# Autodesk Inventor assembly: circuit_boule
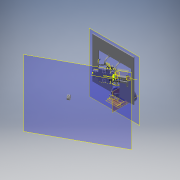
[picture p0: Inventor's stored thumbnail of the model, 180x180]
Saved by Autodesk Inventor 2017 (Build 210142000, 142)
## iProperties
Part Number: circuit_boule
Material: Générique
Document SubType Name: Assembly
Designer: Thomas
Author: Thomas
## Documents named in this file (7)
- C:\Users\Thomas\Documents\Modele 3D\Lanceur boule\circuit_boule.iam
- C:\Users\Thomas\Documents\Modele 3D\Lanceur boule\conduit.ipt
- C:\Users\Thomas\Documents\Modele 3D\Lanceur boule\conduit_bis.ipt
- C:\Users\Thomas\Documents\Modele 3D\Lanceur boule\anneau.ipt
- C:\Users\Thomas\Documents\Modele 3D\Lanceur boule\anneau2.ipt
- C:\Users\Thomas\Documents\Modele 3D\Lanceur boule\Plaque vois.ipt
- C:\Users\Thomas\Documents\Modele 3D\Lanceur boule\Ensemble_Lanceur.iam
## Components (9 placed, 6 different names)
1. conduit:1 — Placage:2, Placage:3
2. conduit_bis:1 — Placage:2, Placage:3
3. anneau:1 — Placage:4
4. anneau:2 — Placage:5
5. anneau2:1 — Placage:6
6. anneau2:2 — Placage:7, Placage:9
7. Plaque vois:1 — Affleurement:1, Placage:4, Placage:5, Placage:6, Placage:7, Placage:10, Affleurement:2
8. anneau2:3 — Placage:9, Placage:10
9. Ensemble_Lanceur:1 [sub-assembly] — Affleurement:2
## Relationships (10: Mate 8, Flush 2)
- Placage:2 [Mate]: conduit:1 ↔ conduit_bis:1
- Placage:3 [Mate]: conduit:1 ↔ conduit_bis:1
- Affleurement:1 [Flush]: Plaque vois:1
- Placage:4 [Mate]: anneau:1 ↔ Plaque vois:1
- Placage:5 [Mate]: anneau:2 ↔ Plaque vois:1
- Placage:6 [Mate]: anneau2:1 ↔ Plaque vois:1
- Placage:7 [Mate]: anneau2:2 ↔ Plaque vois:1
- Placage:9 [Mate] (70 mm): anneau2:2 ↔ anneau2:3
- Placage:10 [Mate]: Plaque vois:1 ↔ anneau2:3
- Affleurement:2 [Flush] (68 mm): Plaque vois:1 ↔ Ensemble_Lanceur:1
